# Autodesk Inventor assembly: RR-PCSS-3M2.ipt
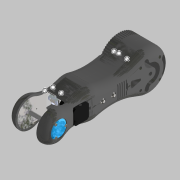
[picture p0: Inventor's stored thumbnail of the model, 180x180]
Saved by Autodesk Inventor 2021 (Build 250183000, 183)
## iProperties
Created: 2021-09-22
Part Number: RR-PCSS-3M2.ipt
Document SubType Name: Assembly
Designer: marci
Author: marci
## Documents named in this file (27)
- C:\Users\marci\Desktop\Projekt ramienia\3M2\RR-PCSS-3M2.ipt.iam
- C:\Users\marci\Desktop\Projekt ramienia\3M2\RR-PCSS-W3M2.ipt
- C:\Users\marci\Desktop\Projekt ramienia\3M2\RR-PCSS-4M1D.ipt
- C:\Users\marci\Desktop\Projekt ramienia\3M2\RR-PCSS-W4M1D.ipt
- C:\Users\marci\Desktop\Projekt ramienia\Nowy folder\pl-PL\ISO 7380-1\ISO 7380-1 - M6 x 12.ipt
- C:\Users\marci\Desktop\Projekt ramienia\Nowy folder\pl-PL\ISO 4161\ISO 4161 - M6(1).ipt
- C:\Users\marci\Desktop\Projekt ramienia\3M2\RR-PCSS-WN.ipt
- C:\Users\marci\Desktop\Projekt ramienia\Nowy folder\pl-PL\ISO 7380-1\ISO 7380-1 - M3 x 6.ipt
- C:\Users\marci\Desktop\Projekt ramienia\3M2\RR-PCSS-MSK.ipt
- C:\Users\marci\Desktop\Projekt ramienia\Nowy folder\pl-PL\ISO 7380-1\ISO 7380-1 - M6 x 10.ipt
- C:\Users\marci\Desktop\Projekt ramienia\3M2\Nema 14.ipt
- C:\Users\marci\Desktop\Projekt ramienia\Nowy folder\pl-PL\ANSI B18.3.1M(1)\ANSI B18.3.1M - M3x0,5 x 35(2).ipt
- C:\Users\marci\Desktop\Projekt ramienia\3M2\M1 Tensor D.iam
- C:\Users\marci\Desktop\Projekt ramienia\3M2\Pulley M5.ipt
- C:\Users\marci\Desktop\Projekt ramienia\3M2\8mm Bearing.ipt
- C:\Users\marci\Desktop\Projekt ramienia\3M2\Barra llisa 8mm x 80mm.ipt
- C:\Users\marci\Desktop\Projekt ramienia\3M2\Tapa 4M1D.ipt
- C:\Users\marci\Desktop\Projekt ramienia\3M2\Tapa 4M1D_MIR.ipt
- C:\Users\marci\Desktop\Projekt ramienia\3M2\RR-PCSS-3M2CC.ipt
- C:\Users\marci\Desktop\Projekt ramienia\Nowy folder\pl-PL\ISO 4762(2)\ISO 4762 - M3 x 8ISO.ipt
- C:\Users\marci\Desktop\Projekt ramienia\3M2\RR-PCSS-3M2C.ipt
- C:\Users\marci\Desktop\Projekt ramienia\Nowy folder\pl-PL\U 2494(1)\Unbrako - M6 x  75(6).ipt
- C:\Users\marci\Desktop\Projekt ramienia\Nowy folder\pl-PL\ISO 4035(2)\ISO 4035 - M6 - ISO.ipt
- C:\Users\marci\Desktop\Projekt ramienia\Nowy folder\pl-PL\U 2494(1)\Unbrako - M3 x  35(6).ipt
- C:\Users\marci\Desktop\Projekt ramienia\Nowy folder\pl-PL\ISO 4035(2)\ISO 4035 - M3 - ISO.ipt
- C:\Users\marci\Desktop\Projekt ramienia\Nowy folder\pl-PL\NF E 25-125\NF E 25-125 - M3 x 16.ipt
- C:\Users\marci\Desktop\Projekt ramienia\Nowy folder\pl-PL\ISO 4762(2)\ISO 4762 - M3 x 16ISO.ipt
## Components (46 placed, 26 different names)
1. RR-PCSS-W3M2:1 — Zestawiające:1, Równoległe:1, Równoległe:2, Zestawiające:21, Zestawiające:23, Zestawiające:25, Zestawiające:26, Zestawiające:27, Zestawiające:28, Zestawiające:40, Zestawiające:42
2. RR-PCSS-W4M1D:1 — Zestawiające:1, Równoległe:1, Równoległe:2, Równoległe:3, Zestawiające:10, Zestawiające:11, Zestawiające:13, Zestawiające:19, Zestawiające:20, Zestawiające:22, Zestawiające:24, Zestawiające:29, Symetria:1
3. ISO 7380-1 M6 x 12:1 — Zestawiające:21, Zestawiające:22
4. ISO 4161 M6:1 — Zestawiające:25, Zestawiające:26
5. RR-PCSS-4M1D:1 — Równoległe:3, Zestawiające:10, Zestawiające:11, Zestawiające:12, Zestawiające:14, Zestawiające:34, Zestawiające:35, Wstawiające:3, Wstawiające:4, Zestawiające:37, Zestawiające:38, Zestawiające:39, Symetria:1, Zestawiające:41
6. RR-PCSS-WN:1 — Zestawiające:12, Zestawiające:13, Zestawiające:14, Zestawiające:15, Zestawiające:16, Zestawiające:17, Zestawiające:18
7. ISO 7380-1 M3 x 6:1 — Zestawiające:15, Zestawiające:16
8. ISO 7380-1 M3 x 6:2 — Zestawiające:17, Zestawiające:18
9. RR-PCSS-MSK:1 — Zestawiające:19, Zestawiające:20, Zestawiające:29, Zestawiające:30, Zestawiające:31, Zestawiające:32, Zestawiające:33, Wstawiające:1, Zestawiające:43, Zestawiające:44, Zestawiające:45, Zestawiające:46, Zestawiające:47, Zestawiające:48, Zestawiające:49, Zestawiające:50
10. ISO 7380-1 M6 x 12:2 — Zestawiające:23, Zestawiające:24
11. ISO 4161 M6:2 — Zestawiające:27, Zestawiające:28
12. ISO 7380-1 M6 x 10:1 — Zestawiające:30, Zestawiające:31
13. ISO 7380-1 M6 x 10:2 — Zestawiające:32, Zestawiające:33
14. Nema 14:1 — Wstawiające:1, Wstawiające:2
15. Wkręt z łbem o zmniejszonych wymiarach z gniazdem ciągnionym - Metryczny M3x0,5 x 35:1 — Zestawiające:34, Zestawiające:35, Zestawiające:36
16. M1 Tensor D:1 [sub-assembly] — Zestawiające:36
17. Pulley M5:1 — Wstawiające:2
18. 8mm Bearing:1 — Wstawiające:4
19. 8mm Bearing:2 — Wstawiające:3, Wstawiające:5
20. Barra llisa 8mm x 80mm:1 — Wstawiające:5
21. Tapa 4M1D:1 — Zestawiające:37, Zestawiające:38, Zestawiające:39, Zestawiające:83, Zestawiające:84, Zestawiające:85, Zestawiające:86, Zestawiające:87, Zestawiające:88
22. Tapa 4M1D_MIR:1 — Zestawiające:77, Zestawiające:78, Zestawiające:79, Zestawiające:80, Zestawiające:81, Zestawiające:82
23. RR-PCSS-3M2CC:1 — Zestawiające:40, Zestawiające:41, Zestawiające:42, Zestawiające:51, Zestawiające:52, Równoległe:4, Zestawiające:61, Zestawiające:62, Zestawiające:63, Zestawiające:64, Zestawiające:65, Zestawiające:66, Zestawiające:67, Zestawiające:68, Zestawiające:69, Zestawiające:71, Zestawiające:73, Zestawiające:75, Zestawiające:89, Zestawiające:90, Zestawiające:91, Zestawiające:92, Zestawiające:93, Zestawiające:95
24. ISO 4762 M3 x 8:1 — Zestawiające:43, Zestawiające:44
25. ISO 4762 M3 x 8:2 — Zestawiające:45, Zestawiające:46
26. ISO 4762 M3 x 8:3 — Zestawiające:47, Zestawiające:48
27. ISO 4762 M3 x 8:4 — Zestawiające:49, Zestawiające:50
28. RR-PCSS-3M2C:1 — Zestawiające:51, Zestawiające:52, Równoległe:4, Zestawiające:70, Zestawiające:72, Zestawiające:74, Zestawiające:76, Zestawiające:94, Zestawiające:96
29. Unbrako Śruba z łbem walcowym z gniazdem sześciokątnym - Metryczny M6 x 75:1 — Zestawiające:89, Zestawiające:90
30. ISO 4035 M6:1 — Zestawiające:93, Zestawiające:94
31. Unbrako Śruba z łbem walcowym z gniazdem sześciokątnym - Metryczny M3 x 35:1 — Zestawiające:61, Zestawiające:62
32. ISO 4035 M3:1 — Zestawiające:69, Zestawiające:70
33. Unbrako Śruba z łbem walcowym z gniazdem sześciokątnym - Metryczny M3 x 35:2 — Zestawiające:63, Zestawiające:64
34. Unbrako Śruba z łbem walcowym z gniazdem sześciokątnym - Metryczny M3 x 35:3 — Zestawiające:65, Zestawiające:66
35. Unbrako Śruba z łbem walcowym z gniazdem sześciokątnym - Metryczny M3 x 35:4 — Zestawiające:67, Zestawiające:68
36. ISO 4035 M3:2 — Zestawiające:71, Zestawiające:72
37. ISO 4035 M3:3 — Zestawiające:73, Zestawiające:74
38. ISO 4035 M3:4 — Zestawiające:75, Zestawiające:76
39. NF E 25-125 M3 x 16:1 — Zestawiające:77, Zestawiające:78
40. NF E 25-125 M3 x 16:2 — Zestawiające:79, Zestawiające:80
41. NF E 25-125 M3 x 16:3 — Zestawiające:81, Zestawiające:82
42. ISO 4762 M3 x 16:1 — Zestawiające:83, Zestawiające:84
43. ISO 4762 M3 x 16:2 — Zestawiające:85, Zestawiające:86
44. ISO 4762 M3 x 16:3 — Zestawiające:87, Zestawiające:88
45. Unbrako Śruba z łbem walcowym z gniazdem sześciokątnym - Metryczny M6 x 75:2 — Zestawiające:91, Zestawiające:92
46. ISO 4035 M6:2 — Zestawiające:95, Zestawiające:96
## Relationships (90: Mate 80, Insert 5, Flush 4, Symmetry 1)
- Zestawiające:1 [Mate]: RR-PCSS-W3M2:1 ↔ RR-PCSS-W4M1D:1
- Równoległe:1 [Flush]: RR-PCSS-W3M2:1 ↔ RR-PCSS-W4M1D:1
- Równoległe:2 [Flush] (-0.1 mm): RR-PCSS-W3M2:1 ↔ RR-PCSS-W4M1D:1
- Równoległe:3 [Flush]: RR-PCSS-W4M1D:1 ↔ RR-PCSS-4M1D:1
- Zestawiające:10 [Mate]: RR-PCSS-W4M1D:1 ↔ RR-PCSS-4M1D:1
- Zestawiające:11 [Mate]: RR-PCSS-W4M1D:1 ↔ RR-PCSS-4M1D:1
- Zestawiające:12 [Mate]: RR-PCSS-4M1D:1 ↔ RR-PCSS-WN:1
- Zestawiające:13 [Mate]: RR-PCSS-W4M1D:1 ↔ RR-PCSS-WN:1
- Zestawiające:14 [Mate]: RR-PCSS-4M1D:1 ↔ RR-PCSS-WN:1
- Zestawiające:15 [Mate]: RR-PCSS-WN:1 ↔ ISO 7380-1 M3 x 6:1
- Zestawiające:16 [Mate]: RR-PCSS-WN:1 ↔ ISO 7380-1 M3 x 6:1
- Zestawiające:17 [Mate]: RR-PCSS-WN:1 ↔ ISO 7380-1 M3 x 6:2
- Zestawiające:18 [Mate]: RR-PCSS-WN:1 ↔ ISO 7380-1 M3 x 6:2
- Zestawiające:19 [Mate]: RR-PCSS-W4M1D:1 ↔ RR-PCSS-MSK:1
- Zestawiające:20 [Mate] (20 mm): RR-PCSS-W4M1D:1 ↔ RR-PCSS-MSK:1
- Zestawiające:21 [Mate]: RR-PCSS-W3M2:1 ↔ ISO 7380-1 M6 x 12:1
- Zestawiające:22 [Mate]: RR-PCSS-W4M1D:1 ↔ ISO 7380-1 M6 x 12:1
- Zestawiające:23 [Mate]: RR-PCSS-W3M2:1 ↔ ISO 7380-1 M6 x 12:2
- Zestawiające:24 [Mate]: RR-PCSS-W4M1D:1 ↔ ISO 7380-1 M6 x 12:2
- Zestawiające:25 [Mate]: RR-PCSS-W3M2:1 ↔ ISO 4161 M6:1
- Zestawiające:26 [Mate]: RR-PCSS-W3M2:1 ↔ ISO 4161 M6:1
- Zestawiające:27 [Mate]: RR-PCSS-W3M2:1 ↔ ISO 4161 M6:2
- Zestawiające:28 [Mate]: RR-PCSS-W3M2:1 ↔ ISO 4161 M6:2
- Zestawiające:29 [Mate] (18.65 mm): RR-PCSS-W4M1D:1 ↔ RR-PCSS-MSK:1
- Zestawiające:30 [Mate]: RR-PCSS-MSK:1 ↔ ISO 7380-1 M6 x 10:1
- Zestawiające:31 [Mate]: RR-PCSS-MSK:1 ↔ ISO 7380-1 M6 x 10:1
- Zestawiające:32 [Mate]: RR-PCSS-MSK:1 ↔ ISO 7380-1 M6 x 10:2
- Zestawiające:33 [Mate]: RR-PCSS-MSK:1 ↔ ISO 7380-1 M6 x 10:2
- Wstawiające:1 [Insert]: RR-PCSS-MSK:1 ↔ Nema 14:1
- Zestawiające:34 [Mate]: RR-PCSS-4M1D:1 ↔ Wkręt z łbem o zmniejszonych wymiarach z gniazdem ciągnionym - Metryczny M3x0,5 x 35:1
- Zestawiające:35 [Mate]: RR-PCSS-4M1D:1 ↔ Wkręt z łbem o zmniejszonych wymiarach z gniazdem ciągnionym - Metryczny M3x0,5 x 35:1
- Zestawiające:36 [Mate]: Wkręt z łbem o zmniejszonych wymiarach z gniazdem ciągnionym - Metryczny M3x0,5 x 35:1 ↔ M1 Tensor D:1
- Wstawiające:2 [Insert] (-2 mm): Nema 14:1 ↔ Pulley M5:1
- Wstawiające:3 [Insert]: RR-PCSS-4M1D:1 ↔ 8mm Bearing:2
- Wstawiające:4 [Insert]: RR-PCSS-4M1D:1 ↔ 8mm Bearing:1
- Wstawiające:5 [Insert]: 8mm Bearing:2 ↔ Barra llisa 8mm x 80mm:1
- Zestawiające:37 [Mate]: RR-PCSS-4M1D:1 ↔ Tapa 4M1D:1
- Zestawiające:38 [Mate]: RR-PCSS-4M1D:1 ↔ Tapa 4M1D:1
- Zestawiające:39 [Mate] (0.528 mm): RR-PCSS-4M1D:1 ↔ Tapa 4M1D:1
- Symetria:1 [Symmetry]: RR-PCSS-W4M1D:1 ↔ RR-PCSS-4M1D:1
- Zestawiające:40 [Mate]: RR-PCSS-W3M2:1 ↔ RR-PCSS-3M2CC:1
- Zestawiające:41 [Mate]: RR-PCSS-4M1D:1 ↔ RR-PCSS-3M2CC:1
- Zestawiające:42 [Mate]: RR-PCSS-W3M2:1 ↔ RR-PCSS-3M2CC:1
- Zestawiające:43 [Mate]: RR-PCSS-MSK:1 ↔ ISO 4762 M3 x 8:1
- Zestawiające:44 [Mate]: RR-PCSS-MSK:1 ↔ ISO 4762 M3 x 8:1
- Zestawiające:45 [Mate]: RR-PCSS-MSK:1 ↔ ISO 4762 M3 x 8:2
- Zestawiające:46 [Mate]: RR-PCSS-MSK:1 ↔ ISO 4762 M3 x 8:2
- Zestawiające:47 [Mate]: RR-PCSS-MSK:1 ↔ ISO 4762 M3 x 8:3
- Zestawiające:48 [Mate]: RR-PCSS-MSK:1 ↔ ISO 4762 M3 x 8:3
- Zestawiające:49 [Mate]: RR-PCSS-MSK:1 ↔ ISO 4762 M3 x 8:4
- Zestawiające:50 [Mate]: RR-PCSS-MSK:1 ↔ ISO 4762 M3 x 8:4
- Zestawiające:51 [Mate]: RR-PCSS-3M2CC:1 ↔ RR-PCSS-3M2C:1
- Zestawiające:52 [Mate]: RR-PCSS-3M2CC:1 ↔ RR-PCSS-3M2C:1
- Równoległe:4 [Flush]: RR-PCSS-3M2CC:1 ↔ RR-PCSS-3M2C:1
- Zestawiające:61 [Mate]: RR-PCSS-3M2CC:1 ↔ Unbrako Śruba z łbem walcowym z gniazdem sześciokątnym - Metryczny M3 x 35:1
- Zestawiające:62 [Mate]: RR-PCSS-3M2CC:1 ↔ Unbrako Śruba z łbem walcowym z gniazdem sześciokątnym - Metryczny M3 x 35:1
- Zestawiające:63 [Mate]: RR-PCSS-3M2CC:1 ↔ Unbrako Śruba z łbem walcowym z gniazdem sześciokątnym - Metryczny M3 x 35:2
- Zestawiające:64 [Mate]: RR-PCSS-3M2CC:1 ↔ Unbrako Śruba z łbem walcowym z gniazdem sześciokątnym - Metryczny M3 x 35:2
- Zestawiające:65 [Mate]: RR-PCSS-3M2CC:1 ↔ Unbrako Śruba z łbem walcowym z gniazdem sześciokątnym - Metryczny M3 x 35:3
- Zestawiające:66 [Mate]: RR-PCSS-3M2CC:1 ↔ Unbrako Śruba z łbem walcowym z gniazdem sześciokątnym - Metryczny M3 x 35:3
- Zestawiające:67 [Mate]: RR-PCSS-3M2CC:1 ↔ Unbrako Śruba z łbem walcowym z gniazdem sześciokątnym - Metryczny M3 x 35:4
- Zestawiające:68 [Mate]: RR-PCSS-3M2CC:1 ↔ Unbrako Śruba z łbem walcowym z gniazdem sześciokątnym - Metryczny M3 x 35:4
- Zestawiające:69 [Mate]: RR-PCSS-3M2CC:1 ↔ ISO 4035 M3:1
- Zestawiające:70 [Mate]: RR-PCSS-3M2C:1 ↔ ISO 4035 M3:1
- Zestawiające:71 [Mate]: RR-PCSS-3M2CC:1 ↔ ISO 4035 M3:2
- Zestawiające:72 [Mate]: RR-PCSS-3M2C:1 ↔ ISO 4035 M3:2
- Zestawiające:73 [Mate]: RR-PCSS-3M2CC:1 ↔ ISO 4035 M3:3
- Zestawiające:74 [Mate]: RR-PCSS-3M2C:1 ↔ ISO 4035 M3:3
- Zestawiające:75 [Mate]: RR-PCSS-3M2CC:1 ↔ ISO 4035 M3:4
- Zestawiające:76 [Mate]: RR-PCSS-3M2C:1 ↔ ISO 4035 M3:4
- Zestawiające:77 [Mate]: Tapa 4M1D_MIR:1 ↔ NF E 25-125 M3 x 16:1
- Zestawiające:78 [Mate]: Tapa 4M1D_MIR:1 ↔ NF E 25-125 M3 x 16:1
- Zestawiające:79 [Mate]: Tapa 4M1D_MIR:1 ↔ NF E 25-125 M3 x 16:2
- Zestawiające:80 [Mate]: Tapa 4M1D_MIR:1 ↔ NF E 25-125 M3 x 16:2
- Zestawiające:81 [Mate]: Tapa 4M1D_MIR:1 ↔ NF E 25-125 M3 x 16:3
- Zestawiające:82 [Mate]: Tapa 4M1D_MIR:1 ↔ NF E 25-125 M3 x 16:3
- Zestawiające:83 [Mate]: Tapa 4M1D:1 ↔ ISO 4762 M3 x 16:1
- Zestawiające:84 [Mate]: Tapa 4M1D:1 ↔ ISO 4762 M3 x 16:1
- Zestawiające:85 [Mate]: Tapa 4M1D:1 ↔ ISO 4762 M3 x 16:2
- Zestawiające:86 [Mate]: Tapa 4M1D:1 ↔ ISO 4762 M3 x 16:2
- Zestawiające:87 [Mate]: Tapa 4M1D:1 ↔ ISO 4762 M3 x 16:3
- Zestawiające:88 [Mate]: Tapa 4M1D:1 ↔ ISO 4762 M3 x 16:3
- Zestawiające:89 [Mate]: RR-PCSS-3M2CC:1 ↔ Unbrako Śruba z łbem walcowym z gniazdem sześciokątnym - Metryczny M6 x 75:1
- Zestawiające:90 [Mate]: RR-PCSS-3M2CC:1 ↔ Unbrako Śruba z łbem walcowym z gniazdem sześciokątnym - Metryczny M6 x 75:1
- Zestawiające:91 [Mate]: RR-PCSS-3M2CC:1 ↔ Unbrako Śruba z łbem walcowym z gniazdem sześciokątnym - Metryczny M6 x 75:2
- Zestawiające:92 [Mate]: RR-PCSS-3M2CC:1 ↔ Unbrako Śruba z łbem walcowym z gniazdem sześciokątnym - Metryczny M6 x 75:2
- Zestawiające:93 [Mate]: RR-PCSS-3M2CC:1 ↔ ISO 4035 M6:1
- Zestawiające:94 [Mate]: RR-PCSS-3M2C:1 ↔ ISO 4035 M6:1
- Zestawiające:95 [Mate]: RR-PCSS-3M2CC:1 ↔ ISO 4035 M6:2
- Zestawiające:96 [Mate]: RR-PCSS-3M2C:1 ↔ ISO 4035 M6:2
